# Autodesk Inventor assembly: __VK_Hubeinehit_100
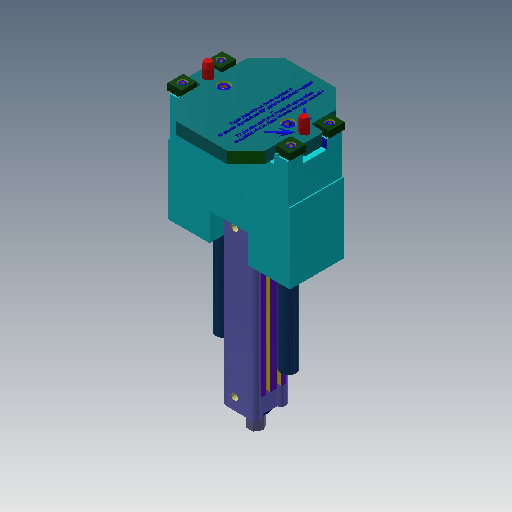
[picture p0: Inventor's stored thumbnail of the model, 512x512]
Saved by Autodesk Inventor 2025.1 (Build 291241000, 241)
## iProperties
Created: 2023-11-18
Part Number: __VK_Hubeinehit_100
Material: Generisch
Document SubType Name: Assembly
Designer: RP
Author: RP
## Documents named in this file (3)
- C:\Users\Erik\Erik\Hochschule\3. Semester\CAD\CAD-Paspa\Useless Box\_Verkettung\__VK_Hubeinehit_100.iam
- C:\Users\Erik\Erik\Hochschule\3. Semester\CAD\CAD-Paspa\Useless Box\_Verkettung\__VK_Hubeinehit_Platform.ipt
- C:\Users\Erik\Erik\Hochschule\3. Semester\CAD\CAD-Paspa\Useless Box\_Verkettung\__VK_Hubeinehit_Führung.ipt
## Components (2 placed, 2 different names)
1. __VK_Hubeinehit_Führung:1 — Passend:1, Passend:2, Passend:3, Passend:4, Fluchtend:2, Fluchtend:3
2. __VK_Hubeinehit_Platform:1 — Passend:1, Passend:2, Passend:3, Fluchtend:4
## Relationships (7: Mate 4, Flush 3)
- Passend:1 [Mate]: __VK_Hubeinehit_Führung:1 ↔ __VK_Hubeinehit_Platform:1
- Passend:2 [Mate]: __VK_Hubeinehit_Führung:1 ↔ __VK_Hubeinehit_Platform:1
- Passend:3 [Mate]: __VK_Hubeinehit_Führung:1 ↔ __VK_Hubeinehit_Platform:1
- Passend:4 [Mate]: __VK_Hubeinehit_Führung:1
- Fluchtend:2 [Flush]: __VK_Hubeinehit_Führung:1
- Fluchtend:3 [Flush] (41.02 mm): __VK_Hubeinehit_Führung:1
- Fluchtend:4 [Flush] (100 mm): __VK_Hubeinehit_Platform:1
